# Autodesk Inventor assembly: Front B
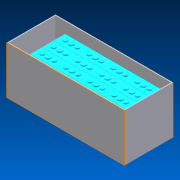
[picture p0: Inventor's stored thumbnail of the model, 180x180]
Saved by Autodesk Inventor 2012 (Build 160160000, 160)
## iProperties
Created: 2012-07-01
Part Number: Front B
Document SubType Name: Assembly
Designer: Hemant
Author: Hemant
## Documents named in this file (3)
- C:\Users\Hemant\Documents\Bat Boxes COmplete\Front B.iam
- C:\Users\Hemant\Documents\medim Battery Box Pastic 2.ipt
- C:\Users\Hemant\Documents\CALB100AH.ipt
## Components (17 placed, 2 different names)
1. medim Battery Box Pastic 2:1 — Mate:1, Mate:2, Mate:3
2. CALB100AH:1
3. CALB100AH:2
4. CALB100AH:3
5. CALB100AH:4
6. CALB100AH:5 — Mate:1
7. CALB100AH:6
8. CALB100AH:7
9. CALB100AH:8
10. CALB100AH:9
11. CALB100AH:10
12. CALB100AH:11
13. CALB100AH:12 — Mate:3
14. CALB100AH:13
15. CALB100AH:14 — Mate:2
16. CALB100AH:15
17. CALB100AH:16
## Component patterns: (4 elements), (4 elements, first: CALB100AH:1), Component Pattern 1:2 (4 elements), Component Pattern 1:3 (4 elements), Component Pattern 1:4 (4 elements)
## Relationships (3: Mate 3)
- Mate:1: medim Battery Box Pastic 2:1 ↔ CALB100AH:5
- Mate:2 (57.15 mm): medim Battery Box Pastic 2:1 ↔ CALB100AH:14
- Mate:3: medim Battery Box Pastic 2:1 ↔ CALB100AH:12
